# Autodesk Inventor assembly: MotorBeltTensioner 10mm
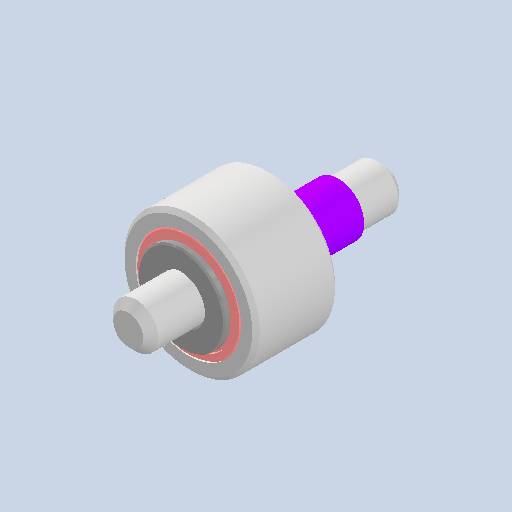
[picture p0: Inventor's stored thumbnail of the model, 512x512]
Saved by Autodesk Inventor 2022.2 (Build 262287000, 287)
## iProperties
Created: 2022-01-06
Part Number: MotorBeltTensioner 10mm
Document SubType Name: Assembly
Designer: Jochen
Author: Jochen
## Documents named in this file (6)
- D:\Projects\Lisbeth\CAD\Common\Belt Tensioner\MotorBeltTensioner 10mm.iam
- D:\Projects\Lisbeth\CAD\Common\Belt Tensioner\MotorBeltTensionerAxis.ipt
- D:\Projects\Lisbeth\CAD\Common\Bearing\bearing_7_3_3_sbn_683_2ZVA.ipt
- D:\Projects\Lisbeth\CAD\Common\Washer\Washer m2.5.ipt
- D:\Projects\Lisbeth\CAD\Common\Belt Tensioner\MotorBeltTensionerRoller 10mm.ipt
- D:\Projects\Lisbeth\CAD\Common\Belt Tensioner\MotorBeltTensionerSleeve 5mm.ipt
## Components (5 placed, 5 different names)
1. MotorBeltTensionerAxis:1 — Mate:9, Mate:18, Mate:21, Mate:22
2. bearing_7_3_3_sbn_683_2ZVA:2 — Mate:9, Mate:16, Mate:17, Mate:20, Mate:21, Mate:23
3. MotorBeltTensionerRoller 10mm:1 — Mate:16, Mate:17
4. MotorBeltTensionerSleeve 6mm:1 — Mate:18, Mate:20
5. Washer m2.5:1 — Mate:22, Mate:23
## Relationships (8: Mate 8)
- Mate:9: MotorBeltTensionerAxis:1 ↔ bearing_7_3_3_sbn_683_2ZVA:2
- Mate:16: bearing_7_3_3_sbn_683_2ZVA:2 ↔ MotorBeltTensionerRoller 10mm:1
- Mate:17: bearing_7_3_3_sbn_683_2ZVA:2 ↔ MotorBeltTensionerRoller 10mm:1
- Mate:18: MotorBeltTensionerAxis:1 ↔ MotorBeltTensionerSleeve 6mm:1
- Mate:20: bearing_7_3_3_sbn_683_2ZVA:2 ↔ MotorBeltTensionerSleeve 6mm:1
- Mate:21 (4 mm): MotorBeltTensionerAxis:1 ↔ bearing_7_3_3_sbn_683_2ZVA:2
- Mate:22: MotorBeltTensionerAxis:1 ↔ Washer m2.5:1
- Mate:23: bearing_7_3_3_sbn_683_2ZVA:2 ↔ Washer m2.5:1
